# Autodesk Inventor assembly: Jack Lift
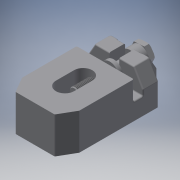
[picture p0: Inventor's stored thumbnail of the model, 180x180]
Saved by Autodesk Inventor 2018 (Build 220112000, 112)
## iProperties
Created: 2019-04-04
Part Number: Jack Lift
Document SubType Name: Assembly
Designer: This kid
Author: This kid
## Documents named in this file (4)
- C:\Users\10043883\Documents\GitHub\IED-files\Jack Lift.iam
- C:\Users\10043883\Desktop\7.0 STUDENTJackLIftInventorFiles\Base.ipt
- C:\Users\10043883\Desktop\7.0 STUDENTJackLIftInventorFiles\Wedge_Screw.ipt
- C:\Users\10043883\Desktop\7.0 STUDENTJackLIftInventorFiles\Wedge.ipt
## Components (3 placed, 3 different names)
1. Base:1 — Mate:1, Mate:2, Flush:1
2. Wedge_Screw:1 — Mate:1, Mate:2
3. Wedge:1 — Flush:1
## Relationships (3: Mate 2, Flush 1)
- Mate:1: Base:1 ↔ Wedge_Screw:1
- Mate:2: Base:1 ↔ Wedge_Screw:1
- Flush:1: Base:1 ↔ Wedge:1
